# Autodesk Inventor assembly: Schlitten
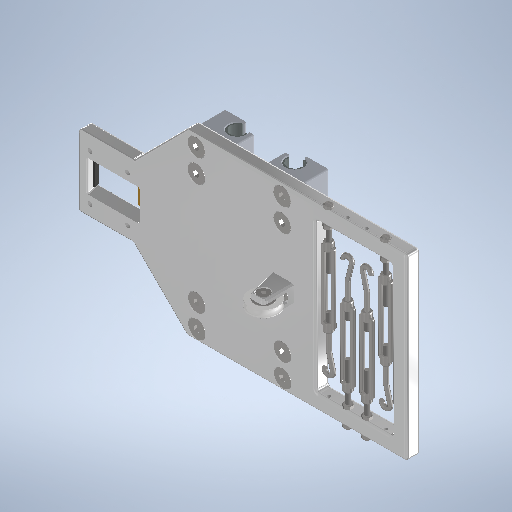
[picture p0: Inventor's stored thumbnail of the model, 512x512]
Saved by Autodesk Inventor 2025 (Build 290162010, 162A)
## iProperties
Created: 2024-11-25
Part Number: Schlitten
Document SubType Name: Assembly
Designer: Admin
Mass: 910.331 g
Surface Area: 1082.39 cm^2
Volume: 241.285 cm^3
Density: 3.77284 g/cm^3
Author: Admin
## Documents named in this file (25)
- C:\Users\Admin\GIT\HDVKBM\CAD\Krandemonstrator\Schlitten.iam
- C:\Users\Admin\GIT\HDVKBM\CAD\Krandemonstrator\SchlittenS.ipt
- C:\Users\Admin\GIT\HDVKBM\CAD\Krandemonstrator\WJ200UM_01_10_1\WJ200UM_01_10_1.iam
- C:\Users\Admin\Documents\Inventor\Content Center Files\R2025\de-DE\DIN 7991(2)\DIN 7991 - M6x16.ipt
- C:\Users\Admin\GIT\HDVKBM\CAD\Krandemonstrator\UmlenkrolleHalterHeavy.iam
- C:\Users\Admin\Documents\Inventor\Content Center Files\R2025\de-DE\DIN 7991(2)\DIN 7991 - M3x10.ipt
- C:\Users\Admin\GIT\HDVKBM\CAD\Krandemonstrator\Bremsbelag.ipt
- C:\Users\Admin\GIT\HDVKBM\CAD\Krandemonstrator\BremsePress.ipt
- C:\Users\Admin\GIT\HDVKBM\CAD\Krandemonstrator\Sliderhalterpress.ipt
- C:\Users\Admin\GIT\HDVKBM\CAD\Krandemonstrator\SchubstangeAPress.ipt
- C:\Users\Admin\GIT\HDVKBM\CAD\Krandemonstrator\SchubstangeAPressB.ipt
- C:\Users\Admin\GIT\HDVKBM\CAD\Krandemonstrator\SliderhalterpressB.ipt
- C:\Users\Admin\GIT\HDVKBM\CAD\Krandemonstrator\Druckfeder15.ipt
- C:\Users\Admin\GIT\HDVKBM\CAD\Krandemonstrator\Druckfeder16.ipt
- C:\Users\Admin\Documents\Inventor\Content Center Files\R2025\de-DE\AS 1427(01)\AS 1427 - M3 x 40(3).ipt
- C:\Users\Admin\GIT\HDVKBM\CAD\Krandemonstrator\Spannschloss M3-wie din1480.ipt
- C:\Users\Admin\GIT\HDVKBM\CAD\Krandemonstrator\M3 Haken 40mm.ipt
- C:\Users\Admin\GIT\HDVKBM\CAD\Krandemonstrator\Zugfeder16.ipt
- C:\Users\Admin\GIT\HDVKBM\CAD\PrintB\BremsbelagBreit.ipt
- C:\Users\Admin\GIT\HDVKBM\CAD\PrintB\Bauteil8.ipt
- C:\Users\Admin\Documents\Inventor\Content Center Files\R2025\de-DE\ISO 2009(1)\ISO 2009 - M2 x 10 - DIN EN 8.ipt
- C:\Users\Admin\Documents\Inventor\Content Center Files\R2025\de-DE\ISO 2009(1)\ISO 2009 - M2 x 5 - DIN EN 3.ipt
- C:\Users\Admin\Documents\Inventor\Content Center Files\R2025\de-DE\ISO 2338(1)\DIN EN ISO 2338 - 2 h8 x 30.ipt
- C:\Users\Admin\Documents\Inventor\Content Center Files\R2025\de-DE\DIN EN ISO 4032\DIN EN ISO 4032 - M3.ipt
- C:\Users\Admin\Documents\Inventor\Content Center Files\R2025\de-DE\ISO 2338(1)\DIN EN ISO 2338 - 2 h8 x 10.ipt
## Components (59 placed, 23 different names)
1. SchlittenS:1 — Passend:1, Passend:2, Passend:3, Passend:4, Starr:17, Starr:15, Starr:18, Starr:16, Planar:6, Drehbar:9, Planar:8, Passend:40, Passend:41, Passend:42, Passend:43, Zylindrisch:40, Zylindrisch:41, Planar:10, Starr:34, Starr:35, Starr:36, Starr:37, Starr:38, Starr:39, Starr:48, Verschiebbar:34, Verschiebbar:32
2. DIN 7991 M3x10:6 — Zylindrisch:41
3. DIN 7991 M3x10:5 — Zylindrisch:40
4. DIN EN ISO 4032 M3:1
5. DIN EN ISO 4032 M3:2
6. DIN EN ISO 4032 M3:3
7. DIN EN ISO 4032 M3:4
8. AS 1427 - Metrisch M3 x 40:4 — Starr:36, Starr:40
9. AS 1427 - Metrisch M3 x 40:1 — Starr:38, Starr:43
10. AS 1427 - Metrisch M3 x 40:2 — Starr:39, Starr:42
11. AS 1427 - Metrisch M3 x 40:3 — Starr:37, Starr:41
12. Spannschloss M3-wie din1480:1 — Starr:40, Starr:45
13. Spannschloss M3-wie din1480:2 — Starr:41, Starr:44
14. Spannschloss M3-wie din1480:3 — Starr:42, Starr:47
15. Spannschloss M3-wie din1480:4 — Starr:43, Starr:46
16. M3 Haken 40mm:1 — Starr:44
17. M3 Haken 40mm:2 — Starr:45
18. M3 Haken 40mm:3 — Starr:46
19. M3 Haken 40mm:4 — Starr:47
20. UmlenkrolleHalterHeavy:1 [sub-assembly] — Planar:10
21. AS 1427 - Metrisch M3 x 40:5 — Starr:31
22. BremsePress:1 — Drehbar:9, Starr:49, Kugelförmig:1
23. DIN EN ISO 2009 M2 x 10:1
24. DIN EN ISO 2009 M2 x 10:2
25. DIN EN ISO 2009 M2 x 5:1
26. DIN EN ISO 2009 M2 x 5:2
27. SchubstangeAPress:1 — Starr:31, Planar:13, Verschiebbar:34
28. SchubstangeAPressB:1 — Verschiebbar:32, Starr:32, Starr:33
29. Druckfeder1:1 — Starr:33
30. Druckfeder1:1 — Starr:32, Planar:13
31. DIN EN ISO 2009 M2 x 10:3
32. DIN EN ISO 2009 M2 x 10:4
33. DIN EN ISO 2338 2 h8 x 30:1 — Starr:48, Zylindrisch:53
34. Zugfeder1:1 — Zylindrisch:53, Starr:51
35. BremsbelagBreit:1 — Starr:49
36. DIN EN ISO 4032 M3:5
37. DIN EN ISO 4032 M3:6
38. Sliderhalterpress:3 — Planar:8
39. DIN EN ISO 2009 M2 x 10:5
40. DIN EN ISO 2009 M2 x 10:6
41. SliderhalterpressB:1 — Planar:6
42. Bauteil8:2 — Verschiebbar:33, Kugelförmig:1
43. Bauteil8:1 — Starr:51, Verschiebbar:33
44. DIN EN ISO 2338 2 h8 x 10:1
45. DIN EN ISO 2338 2 h8 x 10:2
46. WJ200UM_01_10_1:1 [sub-assembly] — Starr:15
47. WJ200UM_01_10_1:2 [sub-assembly] — Starr:16
48. WJ200UM_01_10_1:3 [sub-assembly] — Starr:17
49. WJ200UM_01_10_1:4 [sub-assembly] — Starr:18
50. DIN 7991 M6x16:1 — Passend:1
51. DIN 7991 M6x16:2 — Passend:2
52. DIN 7991 M6x16:3 — Passend:3
53. DIN 7991 M6x16:5 — Passend:40
54. DIN 7991 M6x16:6 — Passend:41
55. DIN 7991 M6x16:7 — Passend:42
56. DIN 7991 M6x16:8 — Passend:43
57. DIN 7991 M6x16:4 — Passend:4
58. Bremsbelag:2 — Starr:34
59. Bremsbelag:1 — Starr:35
## Relationships (77: Mate 30, WeldJoint 26, CylindricalJoint 9, PlanarJoint 4, TranslationJoint 3, RevoluteJoint 2, RelateRotateTranslate 1, RelateRotation 1, BallJoint 1)
- Passend:1 [Mate]: SchlittenS:1 ↔ DIN 7991 M6x16:1
- Passend:2 [Mate]: SchlittenS:1 ↔ DIN 7991 M6x16:2
- Passend:3 [Mate]: SchlittenS:1 ↔ DIN 7991 M6x16:3
- Passend:4 [Mate]: SchlittenS:1 ↔ DIN 7991 M6x16:4
- Starr:17 [WeldJoint]: SchlittenS:1 ↔ WJ200UM_01_10_1:3
- Starr:15 [WeldJoint]: SchlittenS:1 ↔ WJ200UM_01_10_1:1
- Starr:18 [WeldJoint]: SchlittenS:1 ↔ WJ200UM_01_10_1:4
- Starr:16 [WeldJoint]: SchlittenS:1 ↔ WJ200UM_01_10_1:2
- [WeldJoint]: SchlittenS:1 ↔ DIN EN ISO 2338 2 h8 x 10:1
- [WeldJoint]: SchlittenS:1 ↔ DIN EN ISO 2338 2 h8 x 10:2
- [Mate]: DIN 7991 M3x10:5 ↔ UmlenkrolleHalterHeavy:1
- [Mate]: DIN 7991 M3x10:6 ↔ UmlenkrolleHalterHeavy:1
- [Mate]: DIN EN ISO 2009 M2 x 10:5 ↔ SliderhalterpressB:1
- [Mate]: DIN EN ISO 2009 M2 x 10:6 ↔ SliderhalterpressB:1
- Planar:6: SchlittenS:1 ↔ SliderhalterpressB:1
- Drehbar:9 [RevoluteJoint] (0.5 mm): SchlittenS:1 ↔ BremsePress:1
- [Mate]: DIN EN ISO 2009 M2 x 10:1 ↔ Sliderhalterpress:3
- [Mate]: DIN EN ISO 2009 M2 x 10:2 ↔ Sliderhalterpress:3
- [CylindricalJoint]: SchlittenS:1 ↔ DIN EN ISO 2009 M2 x 10:1
- [CylindricalJoint]: SchlittenS:1 ↔ DIN EN ISO 2009 M2 x 10:2
- Planar:8: SchlittenS:1 ↔ Sliderhalterpress:3
- [CylindricalJoint]: SchlittenS:1 ↔ DIN EN ISO 2009 M2 x 10:5
- Starr:31 [WeldJoint] (-2 mm): AS 1427 - Metrisch M3 x 40:5 ↔ SchubstangeAPress:1
- Verschiebbar:32 [TranslationJoint]: SchlittenS:1 ↔ SchubstangeAPressB:1
- Passend:40 [Mate]: SchlittenS:1 ↔ DIN 7991 M6x16:5
- Passend:41 [Mate]: SchlittenS:1 ↔ DIN 7991 M6x16:6
- Passend:42 [Mate]: SchlittenS:1 ↔ DIN 7991 M6x16:7
- Passend:43 [Mate]: SchlittenS:1 ↔ DIN 7991 M6x16:8
- Zylindrisch:40 [CylindricalJoint]: SchlittenS:1 ↔ DIN 7991 M3x10:5
- Zylindrisch:41 [CylindricalJoint]: SchlittenS:1 ↔ DIN 7991 M3x10:6
- Planar:10: SchlittenS:1 ↔ UmlenkrolleHalterHeavy:1
- [CylindricalJoint]: SchlittenS:1 ↔ DIN EN ISO 2009 M2 x 10:6
- Starr:32 [WeldJoint]: SchubstangeAPressB:1 ↔ Druckfeder1:1
- Starr:33 [WeldJoint]: SchubstangeAPressB:1 ↔ Druckfeder1:1
- Planar:13: SchubstangeAPress:1 ↔ Druckfeder1:1
- [Mate]: DIN EN ISO 2009 M2 x 10:3 ↔ SliderhalterpressB:1
- [Mate]: DIN EN ISO 2009 M2 x 10:4 ↔ SliderhalterpressB:1
- [CylindricalJoint]: SchlittenS:1 ↔ DIN EN ISO 2009 M2 x 10:4
- [CylindricalJoint]: SchlittenS:1 ↔ DIN EN ISO 2009 M2 x 10:3
- Starr:34 [WeldJoint]: SchlittenS:1 ↔ Bremsbelag:2
- Starr:35 [WeldJoint]: SchlittenS:1 ↔ Bremsbelag:1
- Starr:36 [WeldJoint]: SchlittenS:1 ↔ AS 1427 - Metrisch M3 x 40:4
- Starr:37 [WeldJoint]: SchlittenS:1 ↔ AS 1427 - Metrisch M3 x 40:3
- Starr:38 [WeldJoint]: SchlittenS:1 ↔ AS 1427 - Metrisch M3 x 40:1
- Starr:39 [WeldJoint]: SchlittenS:1 ↔ AS 1427 - Metrisch M3 x 40:2
- [Mate]: DIN EN ISO 4032 M3:1 ↔ AS 1427 - Metrisch M3 x 40:2
- [Mate]: SchlittenS:1 ↔ DIN EN ISO 4032 M3:1
- [Mate]: DIN EN ISO 4032 M3:2 ↔ AS 1427 - Metrisch M3 x 40:1
- [Mate]: SchlittenS:1 ↔ DIN EN ISO 4032 M3:2
- [Mate]: DIN EN ISO 4032 M3:3 ↔ AS 1427 - Metrisch M3 x 40:4
- [Mate]: SchlittenS:1 ↔ DIN EN ISO 4032 M3:3
- [Mate]: DIN EN ISO 4032 M3:4 ↔ AS 1427 - Metrisch M3 x 40:3
- [Mate]: SchlittenS:1 ↔ DIN EN ISO 4032 M3:4
- Starr:40 [WeldJoint]: AS 1427 - Metrisch M3 x 40:4 ↔ Spannschloss M3-wie din1480:1
- Starr:41 [WeldJoint]: AS 1427 - Metrisch M3 x 40:3 ↔ Spannschloss M3-wie din1480:2
- Starr:42 [WeldJoint]: AS 1427 - Metrisch M3 x 40:2 ↔ Spannschloss M3-wie din1480:3
- Starr:43 [WeldJoint]: AS 1427 - Metrisch M3 x 40:1 ↔ Spannschloss M3-wie din1480:4
- Starr:44 [WeldJoint]: Spannschloss M3-wie din1480:2 ↔ M3 Haken 40mm:1
- Starr:45 [WeldJoint]: Spannschloss M3-wie din1480:1 ↔ M3 Haken 40mm:2
- Starr:46 [WeldJoint]: Spannschloss M3-wie din1480:4 ↔ M3 Haken 40mm:3
- Starr:47 [WeldJoint]: Spannschloss M3-wie din1480:3 ↔ M3 Haken 40mm:4
- [RelateRotateTranslate] (4500 mm): DIN EN ISO 2009 M2 x 10:1 ↔ SchubstangeAPress:1
- [RelateRotation] (1 ul): BremsePress:1 ↔ DIN EN ISO 2009 M2 x 10:1
- Starr:48 [WeldJoint]: SchlittenS:1 ↔ DIN EN ISO 2338 2 h8 x 30:1
- [RevoluteJoint]: DIN EN ISO 2338 2 h8 x 30:1 ↔ Zugfeder1:1
- Starr:49 [WeldJoint]: BremsePress:1 ↔ BremsbelagBreit:1
- [Mate]: AS 1427 - Metrisch M3 x 40:5 ↔ DIN EN ISO 4032 M3:5
- [Mate]: SchubstangeAPress:1 ↔ DIN EN ISO 4032 M3:5
- Zylindrisch:53 [CylindricalJoint]: DIN EN ISO 2338 2 h8 x 30:1 ↔ Zugfeder1:1
- Starr:51 [WeldJoint]: Zugfeder1:1 ↔ Bauteil8:1
- Verschiebbar:33 [TranslationJoint] (0.7 mm): Bauteil8:2 ↔ Bauteil8:1
- Kugelförmig:1 [BallJoint]: BremsePress:1 ↔ Bauteil8:2
- Verschiebbar:34 [TranslationJoint]: SchlittenS:1 ↔ SchubstangeAPress:1
- [Mate]: AS 1427 - Metrisch M3 x 40:5 ↔ DIN EN ISO 4032 M3:6
- [Mate]: AS 1427 - Metrisch M3 x 40:5 ↔ DIN EN ISO 4032 M3:6
- [Mate]: DIN EN ISO 2009 M2 x 5:1 ↔ Sliderhalterpress:3
- [Mate]: DIN EN ISO 2009 M2 x 5:2 ↔ Sliderhalterpress:3
